# Autodesk Inventor assembly: VersaPlanetary 5 to 1 gear kit with ring gear
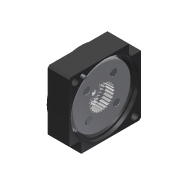
[picture p0: Inventor's stored thumbnail of the model, 180x180]
Saved by Autodesk Inventor 2013 (Build 170138000, 138)
## iProperties
Created: 2013-12-15
Part Number: VersaPlanetary 5 to 1 gear kit with ring gear
Document SubType Name: Assembly
Designer: Nemo
Author: Nemo
## Documents named in this file (4)
- \\lmss\students\Robotics\CAD Files\COTS Parts\VersaPlanetary\VersaPlanetary 5 to 1 Gear Stage.iam
- \\lmss\students\Robotics\CAD Files\COTS Parts\VersaPlanetary\Components\VersaPlanetary Ring Gear.ipt
- \\lmss\students\Robotics\CAD Files\COTS Parts\VersaPlanetary\Components\Gear Stages\VersaPlanetary 5 to 1 gear stage no ring.iam
- \\lmss\students\Robotics\CAD Files\COTS Parts\VersaPlanetary\Components\VersaPlanetary pin.ipt
## Components (3 placed, 3 different names)
1. VersaPlanetary Ring Gear:1 — Mate:1, Flush:1, Insert:1, Mate:2, Flush:2, Mate:3
2. VersaPlanetary 5 to 1 gear stage no ring:1 [sub-assembly] — Mate:1, Flush:1
3. VersaPlanetary pin:1 — Insert:1
## Relationships (6: Mate 3, Flush 2, Insert 1)
- Mate:1: VersaPlanetary Ring Gear:1 ↔ VersaPlanetary 5 to 1 gear stage no ring:1
- Flush:1 (2.032 mm): VersaPlanetary Ring Gear:1 ↔ VersaPlanetary 5 to 1 gear stage no ring:1
- Insert:1: VersaPlanetary Ring Gear:1 ↔ VersaPlanetary pin:1
- Mate:2: VersaPlanetary Ring Gear:1
- Flush:2: VersaPlanetary Ring Gear:1
- Mate:3: VersaPlanetary Ring Gear:1
